# Autodesk Inventor assembly: hand
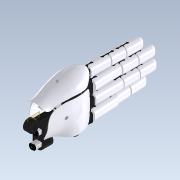
[picture p0: Inventor's stored thumbnail of the model, 180x180]
Saved by Autodesk Inventor 2020.2 (Build 242310000, 310)
## iProperties
Created: 2020-04-08
Part Number: hand
Document SubType Name: Assembly
Designer: Bardo91
thread_hole: 2.500 mm
Author: Bardo91
## Documents named in this file (23)
- D:\programming\elric\hardware\1. hand\elric20-01B.iam
- elric20-01B.iam
- D:\programming\elric\hardware\1. hand\base_hand.ipt
- D:\programming\elric\hardware\1. hand\motor_dc_6v_30rpm.ipt
- D:\programming\elric\hardware\1. hand\finger_pulley.ipt
- D:\programming\elric\hardware\1. hand\cases\hand_case_1.ipt
- D:\programming\elric\hardware\1. hand\cases\hand_case_2.ipt
- D:\programming\elric\hardware\1. hand\cases\hand_case_3.ipt
- D:\programming\elric\hardware\1. hand\potentiometer_bourns_3382_12mm.ipt
- D:\programming\elric\hardware\1. hand\potentiometer_holder.ipt
- D:\programming\elric\hardware\1. hand\index_f1.ipt
- D:\programming\elric\hardware\1. hand\index_f2.ipt
- D:\programming\elric\hardware\1. hand\index_f3.ipt
- D:\programming\elric\hardware\1. hand\index_joint.ipt
- D:\programming\elric\hardware\1. hand\middle_f1.ipt
- D:\programming\elric\hardware\1. hand\middle_f2.ipt
- D:\programming\elric\hardware\1. hand\middle_f3.ipt
- D:\programming\elric\hardware\1. hand\ring_f1.ipt
- D:\programming\elric\hardware\1. hand\ring_f2.ipt
- D:\programming\elric\hardware\1. hand\ring_f3.ipt
- D:\programming\elric\hardware\1. hand\pinky_f1.ipt
- D:\programming\elric\hardware\1. hand\pinky_f2.ipt
- D:\programming\elric\hardware\1. hand\pinky_f3.ipt
## Components (47 placed, 21 different names)
1. base_hand:1 — Mate:78, Flush:18, Mate:79, Mate:80, Mate:81, Mate:83, Mate:84, Mate:85, Mate:87, Mate:88, Mate:89, Mate:92, Mate:93, Mate:94, Mate:95, Mate:96, Flush:19, Flush:20, Mate:98, Mate:99, Mate:100, Mate:102, Mate:103, Angle:1, Angle:2, Angle:3, Mate:116, Flush:26, Mate:122, Flush:27, Mate:128, Flush:38, Mate:134, Flush:44
2. hand_case_1:1
3. hand_case_2:1
4. hand_case_3:1
5. index_joint:12 — Mate:133, Flush:40, Mate:134, Flush:44
6. index_joint:11 — Mate:131, Mate:132, Flush:39, Flush:40, Flush:43
7. index_joint:10 — Mate:129, Mate:130, Flush:39
8. pinky_f2:1 — Mate:130, Mate:131, Flush:41, Flush:42, Flush:43
9. pinky_f3:1 — Mate:129, Flush:42
10. pinky_f1:1 — Mate:132, Mate:133, Flush:41
11. motor_dc_6v_30rpm:2 — Mate:105, Angle:1, Mate:106
12. potentiometer_holder:3 — Tangent:2, Mate:82, Mate:83, Mate:84, Mate:85, Mate:106
13. potentiometer_bourns_3382_12mm:6 — Tangent:2, Mate:82, Mate:105
14. ring_f1:1 — Mate:126, Mate:127, Flush:35
15. ring_f2:1 — Mate:124, Mate:125, Flush:35, Flush:36, Flush:37
16. ring_f3:1 — Mate:123, Flush:36
17. index_joint:7 — Mate:127, Flush:33, Mate:128, Flush:38
18. index_joint:8 — Mate:123, Mate:124, Flush:34, Flush:37
19. index_joint:9 — Mate:125, Mate:126, Flush:33, Flush:34
20. motor_dc_6v_30rpm:1 — Mate:77, Mate:78, Flush:18
21. potentiometer_holder:1 — Mate:79, Mate:80, Mate:81, Tangent:1
22. potentiometer_bourns_3382_12mm:5 — Mate:77, Tangent:1
23. middle_f1:1 — Mate:117, Mate:121, Flush:30
24. middle_f2:1 — Mate:118, Mate:120, Flush:31
25. middle_f3:1 — Mate:119, Flush:32
26. index_joint:4 — Mate:119, Mate:120, Flush:29, Flush:32
27. index_joint:5 — Mate:117, Mate:122, Flush:27, Flush:28, Flush:30
28. index_joint:6 — Mate:118, Mate:121, Flush:28, Flush:29, Flush:31
29. potentiometer_holder:2 — Tangent:3, Mate:86, Mate:87, Mate:88, Mate:89, Mate:110
30. potentiometer_bourns_3382_12mm:3 — Tangent:3, Mate:86, Mate:109
31. motor_dc_6v_30rpm:4 — Angle:3, Mate:109, Mate:110
32. potentiometer_bourns_3382_12mm:1 — Tangent:5, Mate:91, Mate:108
33. index_f1:1 — Mate:111, Mate:112, Flush:23, Flush:25
34. index_f2:1 — Mate:113, Mate:114, Flush:23, Flush:24
35. index_f3:1 — Mate:115, Flush:24
36. index_joint:1 — Mate:111, Flush:21, Flush:25, Mate:116, Flush:26
37. index_joint:2 — Mate:112, Mate:113, Flush:21, Flush:22
38. index_joint:3 — Mate:114, Mate:115, Flush:22
39. potentiometer_holder:5 — Tangent:5, Mate:91, Mate:92, Mate:93, Mate:94, Mate:107
40. motor_dc_6v_30rpm:3 — Mate:107, Mate:108, Angle:2
41. potentiometer_holder:6 — Tangent:6, Mate:101, Mate:102, Mate:103, Mate:104
42. potentiometer_holder:4 — Tangent:4, Mate:90, Mate:98, Mate:99, Mate:100
43. potentiometer_bourns_3382_12mm:4 — Tangent:6, Mate:101
44. potentiometer_bourns_3382_12mm:2 — Tangent:4, Mate:90
45. motor_dc_6v_30rpm:5 — Mate:95, Flush:19
46. motor_dc_6v_30rpm:6 — Mate:67, Mate:68, Mate:96, Flush:20, Mate:104
47. finger_pulley:5 — Mate:67, Mate:68
## Relationships (95: Mate 59, Flush 27, Tangent 6, Angle 3)
- Mate:67: motor_dc_6v_30rpm:6 ↔ finger_pulley:5
- Mate:68 (2.5 mm): motor_dc_6v_30rpm:6 ↔ finger_pulley:5
- Mate:77: motor_dc_6v_30rpm:1 ↔ potentiometer_bourns_3382_12mm:5
- Mate:78: base_hand:1 ↔ motor_dc_6v_30rpm:1
- Flush:18: base_hand:1 ↔ motor_dc_6v_30rpm:1
- Mate:79: base_hand:1 ↔ potentiometer_holder:1
- Mate:80: base_hand:1 ↔ potentiometer_holder:1
- Mate:81: base_hand:1 ↔ potentiometer_holder:1
- Tangent:1: potentiometer_holder:1 ↔ potentiometer_bourns_3382_12mm:5
- Tangent:2: potentiometer_holder:3 ↔ potentiometer_bourns_3382_12mm:6
- Mate:82: potentiometer_holder:3 ↔ potentiometer_bourns_3382_12mm:6
- Mate:83: base_hand:1 ↔ potentiometer_holder:3
- Mate:84: base_hand:1 ↔ potentiometer_holder:3
- Mate:85: base_hand:1 ↔ potentiometer_holder:3
- Tangent:3: potentiometer_holder:2 ↔ potentiometer_bourns_3382_12mm:3
- Mate:86: potentiometer_holder:2 ↔ potentiometer_bourns_3382_12mm:3
- Mate:87: base_hand:1 ↔ potentiometer_holder:2
- Mate:88: base_hand:1 ↔ potentiometer_holder:2
- Mate:89: base_hand:1 ↔ potentiometer_holder:2
- Tangent:4: potentiometer_holder:4 ↔ potentiometer_bourns_3382_12mm:2
- Tangent:5: potentiometer_bourns_3382_12mm:1 ↔ potentiometer_holder:5
- Mate:90: potentiometer_holder:4 ↔ potentiometer_bourns_3382_12mm:2
- Mate:91: potentiometer_bourns_3382_12mm:1 ↔ potentiometer_holder:5
- Mate:92: base_hand:1 ↔ potentiometer_holder:5
- Mate:93: base_hand:1 ↔ potentiometer_holder:5
- Mate:94: base_hand:1 ↔ potentiometer_holder:5
- Mate:95: base_hand:1 ↔ motor_dc_6v_30rpm:5
- Mate:96: base_hand:1 ↔ motor_dc_6v_30rpm:6
- Flush:19: base_hand:1 ↔ motor_dc_6v_30rpm:5
- Flush:20 (5 mm): base_hand:1 ↔ motor_dc_6v_30rpm:6
- Mate:98: base_hand:1 ↔ potentiometer_holder:4
- Mate:99: base_hand:1 ↔ potentiometer_holder:4
- Mate:100: base_hand:1 ↔ potentiometer_holder:4
- Tangent:6: potentiometer_holder:6 ↔ potentiometer_bourns_3382_12mm:4
- Mate:101: potentiometer_holder:6 ↔ potentiometer_bourns_3382_12mm:4
- Mate:102: base_hand:1 ↔ potentiometer_holder:6
- Mate:103: base_hand:1 ↔ potentiometer_holder:6
- Mate:104: potentiometer_holder:6 ↔ motor_dc_6v_30rpm:6
- Mate:105: motor_dc_6v_30rpm:2 ↔ potentiometer_bourns_3382_12mm:6
- Angle:1 (0 deg): base_hand:1 ↔ motor_dc_6v_30rpm:2
- Mate:106: motor_dc_6v_30rpm:2 ↔ potentiometer_holder:3
- Mate:107: potentiometer_holder:5 ↔ motor_dc_6v_30rpm:3
- Mate:108: potentiometer_bourns_3382_12mm:1 ↔ motor_dc_6v_30rpm:3
- Angle:2 (0 deg): base_hand:1 ↔ motor_dc_6v_30rpm:3
- Angle:3 (0 deg): base_hand:1 ↔ motor_dc_6v_30rpm:4
- Mate:109: potentiometer_bourns_3382_12mm:3 ↔ motor_dc_6v_30rpm:4
- Mate:110: potentiometer_holder:2 ↔ motor_dc_6v_30rpm:4
- Mate:111: index_f1:1 ↔ index_joint:1
- Mate:112: index_f1:1 ↔ index_joint:2
- Mate:113: index_f2:1 ↔ index_joint:2
- Mate:114: index_f2:1 ↔ index_joint:3
- Mate:115: index_f3:1 ↔ index_joint:3
- Flush:21: index_joint:1 ↔ index_joint:2
- Flush:22: index_joint:2 ↔ index_joint:3
- Flush:23: index_f1:1 ↔ index_f2:1
- Flush:24: index_f2:1 ↔ index_f3:1
- Flush:25 (1 mm): index_f1:1 ↔ index_joint:1
- Mate:116: base_hand:1 ↔ index_joint:1
- Flush:26 (1 mm): base_hand:1 ↔ index_joint:1
- Mate:117: middle_f1:1 ↔ index_joint:5
- Mate:118: middle_f2:1 ↔ index_joint:6
- Mate:119: middle_f3:1 ↔ index_joint:4
- Mate:120: middle_f2:1 ↔ index_joint:4
- Mate:121: middle_f1:1 ↔ index_joint:6
- Mate:122: base_hand:1 ↔ index_joint:5
- Flush:27 (1 mm): base_hand:1 ↔ index_joint:5
- Flush:28: index_joint:5 ↔ index_joint:6
- Flush:29: index_joint:4 ↔ index_joint:6
- Flush:30 (1 mm): middle_f1:1 ↔ index_joint:5
- Flush:31 (1 mm): middle_f2:1 ↔ index_joint:6
- Flush:32 (1 mm): middle_f3:1 ↔ index_joint:4
- Mate:123: ring_f3:1 ↔ index_joint:8
- Mate:124: ring_f2:1 ↔ index_joint:8
- Mate:125: ring_f2:1 ↔ index_joint:9
- Mate:126: ring_f1:1 ↔ index_joint:9
- Mate:127: ring_f1:1 ↔ index_joint:7
- Flush:33: index_joint:7 ↔ index_joint:9
- Flush:34: index_joint:8 ↔ index_joint:9
- Flush:35: ring_f1:1 ↔ ring_f2:1
- Flush:36: ring_f2:1 ↔ ring_f3:1
- Flush:37 (-1 mm): ring_f2:1 ↔ index_joint:8
- Mate:128: base_hand:1 ↔ index_joint:7
- Flush:38 (-1 mm): base_hand:1 ↔ index_joint:7
- Mate:129: index_joint:10 ↔ pinky_f3:1
- Mate:130: index_joint:10 ↔ pinky_f2:1
- Mate:131: index_joint:11 ↔ pinky_f2:1
- Mate:132: index_joint:11 ↔ pinky_f1:1
- Mate:133: index_joint:12 ↔ pinky_f1:1
- Flush:39: index_joint:11 ↔ index_joint:10
- Flush:40: index_joint:12 ↔ index_joint:11
- Flush:41: pinky_f2:1 ↔ pinky_f1:1
- Flush:42: pinky_f2:1 ↔ pinky_f3:1
- Flush:43 (1 mm): index_joint:11 ↔ pinky_f2:1
- Mate:134: base_hand:1 ↔ index_joint:12
- Flush:44 (1 mm): base_hand:1 ↔ index_joint:12
## Named parameters: thread_hole = 2.5 mm
